# Autodesk Inventor assembly: VerticalParking
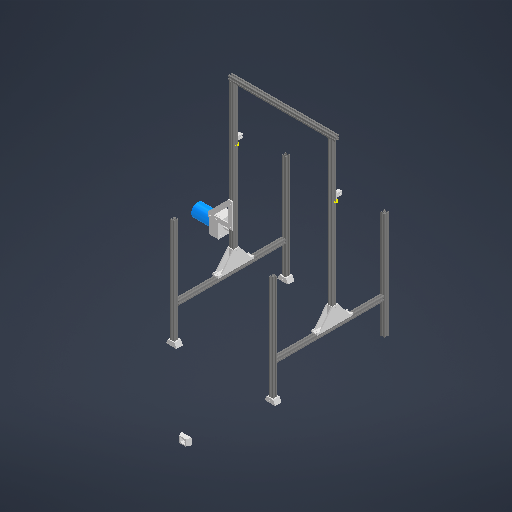
[picture p0: Inventor's stored thumbnail of the model, 512x512]
Saved by Autodesk Inventor 2026.1 (Build 301233020, 233B)
## iProperties
Created: 2025-12-07
Part Number: VerticalParking
Document SubType Name: Assembly
Designer: Tito Luyo Murata
Author: Tito Luyo Murata
## Documents named in this file (9)
- C:\work\verticalparking\diseno3d\VerticalParking.iam
- C:\work\verticalparking\diseno3d\01_Partes\soporte motor.ipt
- C:\work\verticalparking\diseno3d\01_Partes\Escuadra soporte motor.ipt
- C:\work\verticalparking\diseno3d\01_Partes\diseño piezas\motor_v02.ipt
- C:\work\verticalparking\diseno3d\01_Partes\Perfil_Aluminio_20x20x750.ipt
- C:\work\verticalparking\diseno3d\01_Partes\Perfil_Aluminio_20x20x500.ipt
- C:\work\verticalparking\diseno3d\01_Partes\base de soporte.ipt
- C:\work\verticalparking\diseno3d\01_Partes\SoportePrincipal.ipt
- C:\work\verticalparking\diseno3d\01_Partes\diseño piezas\soporte de eje de carril.ipt
## Components (20 placed, 8 different names)
1. soporte motor:1 — Mate:1, Mate:2, Mate:3, Mate:4, Mate:5, Mate:7
2. Escuadra soporte motor:1 — Mate:4, Mate:5, Mate:6, Mate:7, Flush:1, Flush:6
3. motor_v02:1 — Mate:1, Mate:2, Mate:3
4. Perfil_Aluminio_20x20x750:1 — Mate:9, Flush:3, Flush:5, Mate:16, Mate:17, Flush:16, Mate:18, Flush:17, Mate:29, Flush:21, Flush:23
5. Perfil_Aluminio_20x20x750:2 — Mate:6, Flush:1, Mate:8, Flush:2, Flush:4, Flush:6, Mate:14, Mate:15, Flush:15, Mate:19, Flush:19, Mate:30, Flush:22, Flush:24
6. Perfil_Aluminio_20x20x500:1 — Mate:8, Flush:2, Mate:9, Flush:3, Flush:4, Flush:5
7. Perfil_Aluminio_20x20x500:3 — Mate:10, Flush:7, Flush:8, Mate:11, Flush:9, Flush:10, Mate:18, Flush:17, Flush:18
8. Perfil_Aluminio_20x20x500:4 — Mate:11, Flush:9, Flush:10, Mate:26, Mate:27, Mate:28
9. Perfil_Aluminio_20x20x500:5 — Mate:12, Flush:11, Flush:12, Mate:20, Mate:21, Mate:22
10. Perfil_Aluminio_20x20x500:6 — Mate:13, Flush:13, Flush:14, Mate:23, Mate:24, Mate:25
11. Perfil_Aluminio_20x20x500:7 — Mate:10, Flush:7, Flush:8
12. Perfil_Aluminio_20x20x500:8 — Mate:12, Flush:11, Flush:12, Mate:13, Flush:13, Flush:14, Mate:19, Flush:19, Flush:20
13. base de soporte:1
14. base de soporte:2 — Mate:23, Mate:24, Mate:25
15. base de soporte:3 — Mate:26, Mate:27, Mate:28
16. base de soporte:4 — Mate:20, Mate:21, Mate:22
17. SoportePrincipal:1 — Mate:16, Mate:17, Flush:16, Flush:18
18. SoportePrincipal:2 — Mate:14, Mate:15, Flush:15, Flush:20
19. soporte de eje de carril:1 — Mate:29, Flush:21, Flush:23
20. soporte de eje de carril:2 — Mate:30, Flush:22, Flush:24
## Relationships (54: Mate 30, Flush 24)
- Mate:1: soporte motor:1 ↔ motor_v02:1
- Mate:2: soporte motor:1 ↔ motor_v02:1
- Mate:3: soporte motor:1 ↔ motor_v02:1
- Mate:4: soporte motor:1 ↔ Escuadra soporte motor:1
- Mate:5: soporte motor:1 ↔ Escuadra soporte motor:1
- Mate:6: Escuadra soporte motor:1 ↔ Perfil_Aluminio_20x20x750:2
- Mate:7: soporte motor:1 ↔ Escuadra soporte motor:1
- Flush:1: Escuadra soporte motor:1 ↔ Perfil_Aluminio_20x20x750:2
- Mate:8: Perfil_Aluminio_20x20x750:2 ↔ Perfil_Aluminio_20x20x500:1
- Flush:2: Perfil_Aluminio_20x20x750:2 ↔ Perfil_Aluminio_20x20x500:1
- Mate:9: Perfil_Aluminio_20x20x750:1 ↔ Perfil_Aluminio_20x20x500:1
- Flush:3: Perfil_Aluminio_20x20x750:1 ↔ Perfil_Aluminio_20x20x500:1
- Flush:4 (-6.54 mm): Perfil_Aluminio_20x20x750:2 ↔ Perfil_Aluminio_20x20x500:1
- Flush:5 (12.92 mm): Perfil_Aluminio_20x20x750:1 ↔ Perfil_Aluminio_20x20x500:1
- Flush:6 (157 mm): Escuadra soporte motor:1 ↔ Perfil_Aluminio_20x20x750:2
- Mate:10: Perfil_Aluminio_20x20x500:3 ↔ Perfil_Aluminio_20x20x500:7
- Flush:7: Perfil_Aluminio_20x20x500:3 ↔ Perfil_Aluminio_20x20x500:7
- Flush:8 (150 mm): Perfil_Aluminio_20x20x500:3 ↔ Perfil_Aluminio_20x20x500:7
- Mate:11: Perfil_Aluminio_20x20x500:3 ↔ Perfil_Aluminio_20x20x500:4
- Flush:9: Perfil_Aluminio_20x20x500:3 ↔ Perfil_Aluminio_20x20x500:4
- Flush:10 (-150 mm): Perfil_Aluminio_20x20x500:3 ↔ Perfil_Aluminio_20x20x500:4
- Mate:12: Perfil_Aluminio_20x20x500:5 ↔ Perfil_Aluminio_20x20x500:8
- Flush:11: Perfil_Aluminio_20x20x500:5 ↔ Perfil_Aluminio_20x20x500:8
- Flush:12 (150 mm): Perfil_Aluminio_20x20x500:5 ↔ Perfil_Aluminio_20x20x500:8
- Mate:13: Perfil_Aluminio_20x20x500:6 ↔ Perfil_Aluminio_20x20x500:8
- Flush:13: Perfil_Aluminio_20x20x500:6 ↔ Perfil_Aluminio_20x20x500:8
- Flush:14 (150 mm): Perfil_Aluminio_20x20x500:6 ↔ Perfil_Aluminio_20x20x500:8
- Mate:14: Perfil_Aluminio_20x20x750:2 ↔ SoportePrincipal:2
- Mate:15: Perfil_Aluminio_20x20x750:2 ↔ SoportePrincipal:2
- Flush:15: Perfil_Aluminio_20x20x750:2 ↔ SoportePrincipal:2
- Mate:16: Perfil_Aluminio_20x20x750:1 ↔ SoportePrincipal:1
- Mate:17: Perfil_Aluminio_20x20x750:1 ↔ SoportePrincipal:1
- Flush:16: Perfil_Aluminio_20x20x750:1 ↔ SoportePrincipal:1
- Mate:18: Perfil_Aluminio_20x20x750:1 ↔ Perfil_Aluminio_20x20x500:3
- Flush:17: Perfil_Aluminio_20x20x750:1 ↔ Perfil_Aluminio_20x20x500:3
- Flush:18 (150 mm): Perfil_Aluminio_20x20x500:3 ↔ SoportePrincipal:1
- Mate:19: Perfil_Aluminio_20x20x750:2 ↔ Perfil_Aluminio_20x20x500:8
- Flush:19: Perfil_Aluminio_20x20x750:2 ↔ Perfil_Aluminio_20x20x500:8
- Flush:20 (150 mm): Perfil_Aluminio_20x20x500:8 ↔ SoportePrincipal:2
- Mate:20: Perfil_Aluminio_20x20x500:5 ↔ base de soporte:4
- Mate:21: Perfil_Aluminio_20x20x500:5 ↔ base de soporte:4
- Mate:22: Perfil_Aluminio_20x20x500:5 ↔ base de soporte:4
- Mate:23: Perfil_Aluminio_20x20x500:6 ↔ base de soporte:2
- Mate:24: Perfil_Aluminio_20x20x500:6 ↔ base de soporte:2
- Mate:25: Perfil_Aluminio_20x20x500:6 ↔ base de soporte:2
- Mate:26: Perfil_Aluminio_20x20x500:4 ↔ base de soporte:3
- Mate:27: Perfil_Aluminio_20x20x500:4 ↔ base de soporte:3
- Mate:28: Perfil_Aluminio_20x20x500:4 ↔ base de soporte:3
- Mate:29: Perfil_Aluminio_20x20x750:1 ↔ soporte de eje de carril:1
- Flush:21 (2.5 mm): Perfil_Aluminio_20x20x750:1 ↔ soporte de eje de carril:1
- Mate:30: Perfil_Aluminio_20x20x750:2 ↔ soporte de eje de carril:2
- Flush:22 (-2.5 mm): Perfil_Aluminio_20x20x750:2 ↔ soporte de eje de carril:2
- Flush:23 (215 mm): Perfil_Aluminio_20x20x750:1 ↔ soporte de eje de carril:1
- Flush:24 (215 mm): Perfil_Aluminio_20x20x750:2 ↔ soporte de eje de carril:2
